# Autodesk Inventor assembly: roda_boba
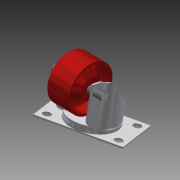
[picture p0: Inventor's stored thumbnail of the model, 180x180]
Saved by Autodesk Inventor 2014 (Build 180170000, 170)
## iProperties
Created: 2015-06-10
Part Number: roda_boba
Document SubType Name: Assembly
Designer: Gabriel
Author: Gabriel
## Documents named in this file (5)
- C:\Users\Gabriel\Desktop\Esboço_robô\rodabobagrande\roda_boba.iam
- C:\Users\Gabriel\Desktop\Esboço_robô\rodabobagrande\sup_rodaboba2.ipt
- C:\Users\Gabriel\Desktop\Esboço_robô\rodabobagrande\apoiorodaboba2.ipt
- C:\Users\Gabriel\Desktop\Esboço_robô\rodabobagrande\eixorodaboba2.ipt
- C:\Users\Gabriel\Desktop\Esboço_robô\rodabobagrande\rodaboba2.ipt
## Components (4 placed, 4 different names)
1. sup_rodaboba2:1 — Rotational:1
2. apoiorodaboba2:1 — Rotational:1, Cylindrical:1
3. eixorodaboba2:1 — Cylindrical:1, Cylindrical:2
4. rodaboba2:1 — Cylindrical:2
## Relationships (3: CylindricalJoint 2, RevoluteJoint 1)
- Rotational:1 [RevoluteJoint]: sup_rodaboba2:1 ↔ apoiorodaboba2:1
- Cylindrical:1: apoiorodaboba2:1 ↔ eixorodaboba2:1
- Cylindrical:2: eixorodaboba2:1 ↔ rodaboba2:1
